# Autodesk Inventor assembly: ankle_w_motor_fin1_opp
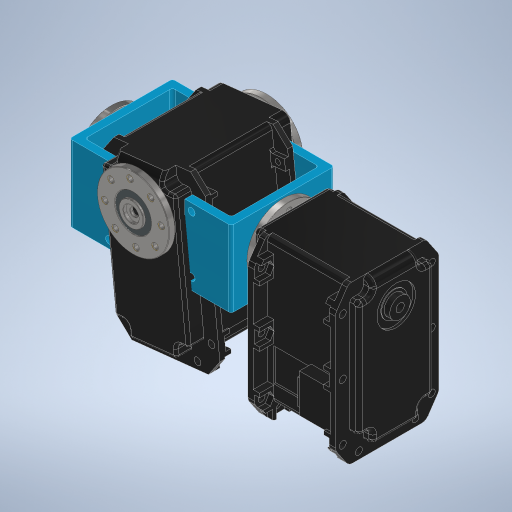
[picture p0: Inventor's stored thumbnail of the model, 512x512]
Saved by Autodesk Inventor 2024 (Build 280153000, 153)
## iProperties
Created: 2024-09-14
Part Number: ankle_w_motor_fin1_opp
Document SubType Name: Assembly
Designer: jmha0
Author: jmha0
## Documents named in this file (8)
- C:\Users\jmha0\OneDrive\바탕 화면\19th_intern_hjm_fight_robot\Lower_Body\ankle_w_motor\ankle_w_motor_fin1_opp.iam
- C:\Users\jmha0\OneDrive\바탕 화면\19th_intern_hjm_fight_robot\hardware\ROBOTIS(Inventor 2024 ver.)\다이나믹셀\MX-106T+idle.ipt.iam
- C:\Users\jmha0\OneDrive\바탕 화면\19th_intern_hjm_fight_robot\hardware\ROBOTIS(Inventor 2024 ver.)\혼\64-106Horn.ipt
- C:\Users\jmha0\OneDrive\바탕 화면\19th_intern_hjm_fight_robot\Lower_Body\ankle_w_motor\3D_ankle1.ipt
- C:\Users\jmha0\OneDrive\바탕 화면\19th_intern_hjm_fight_robot\Lower_Body\ankle_w_motor\3D_ankle2.ipt
- C:\Users\jmha0\OneDrive\바탕 화면\19th_intern_hjm_fight_robot\hardware\ROBOTIS(Inventor 2024 ver.)\아이들러\64아이들러.iam
- C:\Users\jmha0\OneDrive\바탕 화면\19th_intern_hjm_fight_robot\hardware\ROBOTIS(Inventor 2024 ver.)\다이나믹셀\MX-64T.ipt
- MX-106T+idle.ipt
## Components (7 placed, 6 different names)
1. MX-106T+idle.ipt:1 [sub-assembly] — 삽입:16, 삽입:17, 삽입:18
2. 64-106Horn:1
3. 3D_ankle1:1 — 삽입:16, 삽입:18
4. 3D_ankle2:1 — 삽입:17
5. 64아이들러:1 [sub-assembly]
6. MX-64T:1
7. 64-106Horn:2
## Relationships (10: Insert 10)
- [Insert] (0.1 mm): MX-106T+idle.ipt:1 ↔ 64-106Horn:1
- [Insert] (0.1 mm): 3D_ankle1:1 ↔ 64아이들러:1
- [Insert] (0.1 mm): MX-64T:1 ↔ 64-106Horn:2
- [Insert]: 3D_ankle2:1 ↔ 64-106Horn:2
- [Insert]: 3D_ankle2:1 ↔ 64-106Horn:2
- [Insert]: 3D_ankle2:1 ↔ 64-106Horn:2
- [Insert]: 3D_ankle2:1 ↔ 64-106Horn:2
- 삽입:16 [Insert]: MX-106T+idle.ipt:1 ↔ 3D_ankle1:1
- 삽입:17 [Insert]: MX-106T+idle.ipt:1 ↔ 3D_ankle2:1
- 삽입:18 [Insert]: MX-106T+idle.ipt:1 ↔ 3D_ankle1:1
## Named parameters: d11_d12 = 0 mm, d12_d13 = 0 mm, d13_d14 = 0 mm
